# Autodesk Inventor assembly: Arm Assembly 2
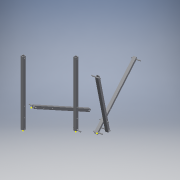
[picture p0: Inventor's stored thumbnail of the model, 180x180]
Saved by Autodesk Inventor 2016 (Build 200138000, 138)
## iProperties
Created: 2016-02-05
Part Number: Arm Assembly 2
Document SubType Name: Assembly
Designer: gus
Author: gus
## Documents named in this file (3)
- \\Mac\Home\Desktop\1510-stronghold-CAD-master\roller cage\Arm Assembly 2.iam
- \\Mac\Home\Desktop\1510-stronghold-CAD-master\roller cage\26 inch 8th inch thick tube.ipt
- \\Mac\Home\Desktop\1510-stronghold-CAD-master\roller cage\3 inch bolt.ipt
## Components (12 placed, 2 different names)
1. 26 inch 8th inch thick tube:1 — Rotational:2, Rotational:6, Rotational:7, Rotational:8
2. 26 inch 8th inch thick tube:2 — Rotational:1, Rotational:5, Rotational:8
3. 26 inch 8th inch thick tube:3 — Rotational:3
4. 26 inch 8th inch thick tube:4
5. 3 inch bolt:1 — Rotational:3
6. 3 inch bolt:2 — Rotational:2
7. 3 inch bolt:3 — Rotational:5
8. 3 inch bolt:4 — Rotational:1
9. 3 inch bolt:5 — Rotational:7
10. 3 inch bolt:6 — Rotational:6
11. 3 inch bolt:7
12. 26 inch 8th inch thick tube:5
## Relationships (7: RevoluteJoint 7)
- Rotational:1 [RevoluteJoint]: 26 inch 8th inch thick tube:2 ↔ 3 inch bolt:4
- Rotational:2 [RevoluteJoint]: 26 inch 8th inch thick tube:1 ↔ 3 inch bolt:2
- Rotational:3 [RevoluteJoint]: 26 inch 8th inch thick tube:3 ↔ 3 inch bolt:1
- Rotational:5 [RevoluteJoint]: 26 inch 8th inch thick tube:2 ↔ 3 inch bolt:3
- Rotational:6 [RevoluteJoint]: 26 inch 8th inch thick tube:1 ↔ 3 inch bolt:6
- Rotational:7 [RevoluteJoint]: 26 inch 8th inch thick tube:1 ↔ 3 inch bolt:5
- Rotational:8 [RevoluteJoint]: 26 inch 8th inch thick tube:1 ↔ 26 inch 8th inch thick tube:2
